# Autodesk Inventor assembly: SF87_20210618_214211_
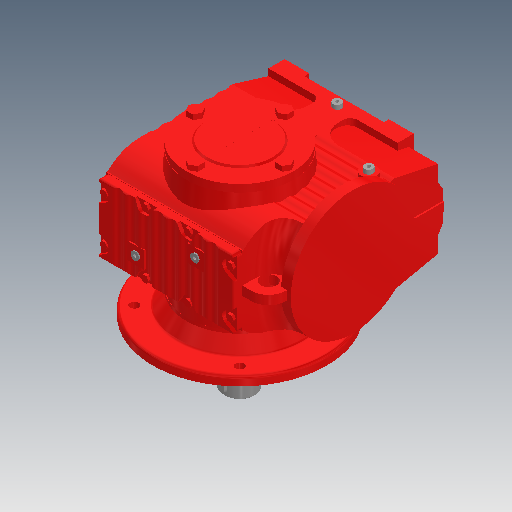
[picture p0: Inventor's stored thumbnail of the model, 512x512]
Saved by Autodesk Inventor 2021 (Build 250183000, 183)
## iProperties
Company: CADClick - www.CADClick.com
Created: 2021-06-18
Part Number: SF87_20210618_214211_
Description: STEP AP214
Document SubType Name: Assembly
Designer: Andrés Holguín
Authority: unknown authorization
Preprocessor: Spatial InterOp 3D postprocessed
Title: cctmp_877BB0B1-044A-4A39-9526-89BE42DB34D8_2021_6_18_21_42_15_205..stp
Author: SEW-EURODRIVE GmbH & Co KG
Revision Number: NONE
## Documents named in this file (13)
- C:\Users\Santiago Suárez\Documents\GitHub\Dis.-Mecatronico-E6\inventor proyecto\Motores y reductores\Reductor Izquierda.iam
- C:\Users\Santiago Suárez\Documents\GitHub\Dis.-Mecatronico-E6\inventor proyecto\Motores y reductores\2021_06_18__21-42-15-174.ipt
- C:\Users\Santiago Suárez\Documents\GitHub\Dis.-Mecatronico-E6\inventor proyecto\Motores y reductores\2021_06_18__21-42-15-142.ipt
- C:\Users\Santiago Suárez\Documents\GitHub\Dis.-Mecatronico-E6\inventor proyecto\Motores y reductores\2021_06_18__21-42-15-111.ipt
- C:\Users\Santiago Suárez\Documents\GitHub\Dis.-Mecatronico-E6\inventor proyecto\Motores y reductores\2021_06_18__21-42-15-080.ipt
- C:\Users\Santiago Suárez\Documents\GitHub\Dis.-Mecatronico-E6\inventor proyecto\Motores y reductores\2021_06_18__21-42-15-049.ipt
- C:\Users\Santiago Suárez\Documents\GitHub\Dis.-Mecatronico-E6\inventor proyecto\Motores y reductores\2021_06_18__21-42-15-017.ipt
- C:\Users\Santiago Suárez\Documents\GitHub\Dis.-Mecatronico-E6\inventor proyecto\Motores y reductores\2021_06_18__21-42-14-986.ipt
- C:\Users\Santiago Suárez\Documents\GitHub\Dis.-Mecatronico-E6\inventor proyecto\Motores y reductores\2021_06_18__21-42-14-955.ipt
- C:\Users\Santiago Suárez\Documents\GitHub\Dis.-Mecatronico-E6\inventor proyecto\Motores y reductores\2021_06_18__21-42-14-924.ipt
- C:\Users\Santiago Suárez\Documents\GitHub\Dis.-Mecatronico-E6\inventor proyecto\Motores y reductores\2021_06_18__21-42-14-892.ipt
- C:\Users\Santiago Suárez\Documents\GitHub\Dis.-Mecatronico-E6\inventor proyecto\Motores y reductores\2021_06_18__21-42-14-861.ipt
- C:\Users\Santiago Suárez\Documents\GitHub\Dis.-Mecatronico-E6\inventor proyecto\Motores y reductores\2021_06_18__21-42-14-830.ipt
## Components (12 placed, 12 different names)
1. 2021_06_18__21-42-15-174 — Rigid:1, Rotational:4, Rotational:5, Rigid:2, Rotational:6, Rotational:7, Rotational:8, Rigid:3
2. 2021_06_18__21-42-15-142 — Rotational:5
3. 2021_06_18__21-42-15-111 — Rotational:8
4. 2021_06_18__21-42-15-080 — Rotational:7
5. 2021_06_18__21-42-15-049 — Rotational:4
6. 2021_06_18__21-42-15-017 — Rotational:6
7. 2021_06_18__21-42-14-986 — Rigid:2
8. 2021_06_18__21-42-14-955 — Rigid:3, Insert:1
9. 2021_06_18__21-42-14-924 — Insert:1
10. 2021_06_18__21-42-14-892 — Rotational:2, Rotational:3, Rigid:1
11. 2021_06_18__21-42-14-861 — Rotational:2
12. 2021_06_18__21-42-14-830 — Rotational:3
## Relationships (11: RevoluteJoint 7, WeldJoint 3, Insert 1)
- Rotational:2 [RevoluteJoint]: 2021_06_18__21-42-14-892 ↔ 2021_06_18__21-42-14-861
- Rotational:3 [RevoluteJoint]: 2021_06_18__21-42-14-892 ↔ 2021_06_18__21-42-14-830
- Rigid:1 [WeldJoint]: 2021_06_18__21-42-15-174 ↔ 2021_06_18__21-42-14-892
- Rotational:4 [RevoluteJoint]: 2021_06_18__21-42-15-174 ↔ 2021_06_18__21-42-15-049
- Rotational:5 [RevoluteJoint]: 2021_06_18__21-42-15-174 ↔ 2021_06_18__21-42-15-142
- Rigid:2 [WeldJoint]: 2021_06_18__21-42-15-174 ↔ 2021_06_18__21-42-14-986
- Rotational:6 [RevoluteJoint]: 2021_06_18__21-42-15-174 ↔ 2021_06_18__21-42-15-017
- Rotational:7 [RevoluteJoint]: 2021_06_18__21-42-15-174 ↔ 2021_06_18__21-42-15-080
- Rotational:8 [RevoluteJoint]: 2021_06_18__21-42-15-174 ↔ 2021_06_18__21-42-15-111
- Rigid:3 [WeldJoint]: 2021_06_18__21-42-15-174 ↔ 2021_06_18__21-42-14-955
- Insert:1: 2021_06_18__21-42-14-955 ↔ 2021_06_18__21-42-14-924
